# Autodesk Inventor assembly: MGSE_Lateral
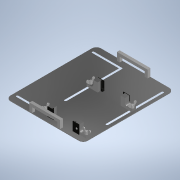
[picture p0: Inventor's stored thumbnail of the model, 180x180]
Saved by Autodesk Inventor 2022 (Build 260153000, 153)
## iProperties
Part Number: MGSE_Lateral
Document SubType Name: Assembly
Designer: braxt
Author: braxt
## Documents named in this file (11)
- C:\Users\braxt\Documents\Vault\Engineering Data\MemeSat\MGSE\v2\MGSE_Lateral.iam
- C:\Users\braxt\Documents\Vault\Engineering Data\MemeSat\MGSE\v2\PlateLateral.ipt
- C:\Users\braxt\Documents\Vault\Engineering Data\MemeSat\MGSE\v2\Bracket_Short.ipt
- C:\Users\braxt\Documents\Vault\Engineering Data\MemeSat\MGSE\v2\Bracket_Short2.ipt
- C:\Users\braxt\Documents\Vault\Engineering Data\MemeSat\MGSE\v2\3DPrintBracket.ipt
- C:\Users\braxt\Documents\Vault\Engineering Data\MemeSat\MGSE\v2\3DPrintBracket2.ipt
- C:\Users\braxt\Documents\Vault\Content Center Files\en-US\IFI 513(1)\IFI 513 - M4x0.7 x 10(1) I.ipt
- C:\Users\braxt\Documents\Vault\Content Center Files\en-US\DIN 315\DIN 315 - M8.ipt
- C:\Users\braxt\Documents\Vault\Content Center Files\en-US\DIN 933\DIN 933 - M8  x 22.ipt
- C:\Users\braxt\Documents\Vault\Engineering Data\MemeSat\MGSE\v2\BarHandle5in.ipt
- C:\Users\braxt\Documents\Vault\Content Center Files\en-US\ANSI B18.6.3(24)\ANSI B18.6.3 - 12-24 UNC - 1(4A).ipt
## Components (27 placed, 10 different names)
1. PlateLateral:1 — Mate:2, Mate:3, Mate:4, Mate:5, Mate:7, Mate:33, Mate:34, Mate:40, Mate:41, Mate:42, Mate:44, Mate:46, Mate:48, Mate:49
2. Bracket_Short:1 — Mate:2, Mate:3, Mate:4, Mate:8, Mate:9
3. Bracket_Short2:1 — Mate:12, Mate:21, Mate:33, Mate:34
4. Bracket_Short:2 — Mate:5, Mate:11
5. Bracket_Short2:2 — Mate:7, Mate:8, Mate:10
6. 3DPrintBracket:1 — Mate:9, Mate:32
7. 3DPrintBracket2:1 — Mate:12, Mate:30
8. 3DPrintBracket:2 — Mate:11, Mate:29
9. 3DPrintBracket2:2 — Mate:10, Mate:31
10. DIN 933 - replaced by DIN EN 24017 M8  x 22:1
11. DIN 315 M8:1
12. DIN 933 - replaced by DIN EN 24017 M8  x 22:2
13. DIN 315 M8:2
14. DIN 933 - replaced by DIN EN 24017 M8  x 22:3 — Mate:21, Insert:1, Mate:35
15. DIN 315 M8:3 — Insert:1, Mate:35
16. DIN 933 - replaced by DIN EN 24017 M8  x 22:4
17. DIN 315 M8:4
18. Cross Recessed Flat Countersunk Head Machine Screw - Type I - Metric M4x0.7 x 10:1 — Mate:29
19. Cross Recessed Flat Countersunk Head Machine Screw - Type I - Metric M4x0.7 x 10:2 — Mate:30
20. Cross Recessed Flat Countersunk Head Machine Screw - Type I - Metric M4x0.7 x 10:3 — Mate:31
21. Cross Recessed Flat Countersunk Head Machine Screw - Type I - Metric M4x0.7 x 10:4 — Mate:32
22. BarHandle5in:1 — Mate:40, Mate:42, Mate:43, Mate:45
23. BarHandle5in:2 — Mate:41, Mate:47, Mate:48
24. Cross Recessed Pan Head Machine Screw - Type I - Inch No. 12 - 24 - 1:1 — Mate:43, Mate:44, Mate:45
25. Cross Recessed Pan Head Machine Screw - Type I - Inch No. 12 - 24 - 1:2 — Mate:46
26. Cross Recessed Pan Head Machine Screw - Type I - Inch No. 12 - 24 - 1:3 — Mate:47
27. Cross Recessed Pan Head Machine Screw - Type I - Inch No. 12 - 24 - 1:4 — Mate:49
## Relationships (43: Mate 42, Insert 1)
- Mate:2 (5 mm): PlateLateral:1 ↔ Bracket_Short:1
- Mate:3 (5 mm): PlateLateral:1 ↔ Bracket_Short:1
- Mate:4: PlateLateral:1 ↔ Bracket_Short:1
- Mate:5: PlateLateral:1 ↔ Bracket_Short:2
- Mate:7: PlateLateral:1 ↔ Bracket_Short2:2
- Mate:8 (104 mm): Bracket_Short:1 ↔ Bracket_Short2:2
- Mate:9: Bracket_Short:1 ↔ 3DPrintBracket:1
- Mate:10: Bracket_Short2:2 ↔ 3DPrintBracket2:2
- Mate:11: Bracket_Short:2 ↔ 3DPrintBracket:2
- Mate:12: Bracket_Short2:1 ↔ 3DPrintBracket2:1
- [Mate]: Bracket_Short2:2 ↔ DIN 933 - replaced by DIN EN 24017 M8  x 22:1
- [Mate] (1.175 mm): Bracket_Short2:2 ↔ DIN 933 - replaced by DIN EN 24017 M8  x 22:1
- [Mate]: Bracket_Short2:2 ↔ DIN 315 M8:1
- [Mate]: Bracket_Short2:2 ↔ DIN 315 M8:1
- [Mate]: Bracket_Short:2 ↔ DIN 933 - replaced by DIN EN 24017 M8  x 22:2
- [Mate] (1.175 mm): Bracket_Short:2 ↔ DIN 933 - replaced by DIN EN 24017 M8  x 22:2
- [Mate]: Bracket_Short:2 ↔ DIN 315 M8:2
- [Mate]: Bracket_Short:2 ↔ DIN 315 M8:2
- Mate:21: Bracket_Short2:1 ↔ DIN 933 - replaced by DIN EN 24017 M8  x 22:3
- [Mate] (1.175 mm): Bracket_Short2:1 ↔ DIN 933 - replaced by DIN EN 24017 M8  x 22:3
- [Mate]: Bracket_Short2:1 ↔ DIN 315 M8:3
- [Mate]: Bracket_Short:1 ↔ DIN 933 - replaced by DIN EN 24017 M8  x 22:4
- [Mate] (1.175 mm): Bracket_Short:1 ↔ DIN 933 - replaced by DIN EN 24017 M8  x 22:4
- [Mate]: Bracket_Short:1 ↔ DIN 315 M8:4
- [Mate]: Bracket_Short:1 ↔ DIN 315 M8:4
- Mate:29: 3DPrintBracket:2 ↔ Cross Recessed Flat Countersunk Head Machine Screw - Type I - Metric M4x0.7 x 10:1
- Mate:30: 3DPrintBracket2:1 ↔ Cross Recessed Flat Countersunk Head Machine Screw - Type I - Metric M4x0.7 x 10:2
- Mate:31: 3DPrintBracket2:2 ↔ Cross Recessed Flat Countersunk Head Machine Screw - Type I - Metric M4x0.7 x 10:3
- Mate:32: 3DPrintBracket:1 ↔ Cross Recessed Flat Countersunk Head Machine Screw - Type I - Metric M4x0.7 x 10:4
- Mate:33: PlateLateral:1 ↔ Bracket_Short2:1
- Mate:34: PlateLateral:1 ↔ Bracket_Short2:1
- Insert:1: DIN 933 - replaced by DIN EN 24017 M8  x 22:3 ↔ DIN 315 M8:3
- Mate:35: DIN 933 - replaced by DIN EN 24017 M8  x 22:3 ↔ DIN 315 M8:3
- Mate:40: PlateLateral:1 ↔ BarHandle5in:1
- Mate:41: PlateLateral:1 ↔ BarHandle5in:2
- Mate:42: PlateLateral:1 ↔ BarHandle5in:1
- Mate:43: BarHandle5in:1 ↔ Cross Recessed Pan Head Machine Screw - Type I - Inch No. 12 - 24 - 1:1
- Mate:44: PlateLateral:1 ↔ Cross Recessed Pan Head Machine Screw - Type I - Inch No. 12 - 24 - 1:1
- Mate:45: BarHandle5in:1 ↔ Cross Recessed Pan Head Machine Screw - Type I - Inch No. 12 - 24 - 1:1
- Mate:46: PlateLateral:1 ↔ Cross Recessed Pan Head Machine Screw - Type I - Inch No. 12 - 24 - 1:2
- Mate:47: BarHandle5in:2 ↔ Cross Recessed Pan Head Machine Screw - Type I - Inch No. 12 - 24 - 1:3
- Mate:48: PlateLateral:1 ↔ BarHandle5in:2
- Mate:49: PlateLateral:1 ↔ Cross Recessed Pan Head Machine Screw - Type I - Inch No. 12 - 24 - 1:4
